# Autodesk Inventor assembly: Сборка всего
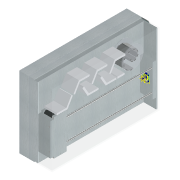
[picture p0: Inventor's stored thumbnail of the model, 180x180]
Saved by Autodesk Inventor 2022 (Build 260153000, 153)
## iProperties
Created: 2023-02-18
Part Number: Сборка всего
Document SubType Name: Assembly
Designer: Глеб
Mass: 16857.9 g
Surface Area: 28110.4 cm^2
Volume: 16853.6 cm^3
Density: 1.00025 g/cm^3
Author: Глеб
## Documents named in this file (12)
- C:\Users\Глеб\Documents\Inventor\Файлы Inventor\Сборка всего.iam
- C:\Users\Глеб\Documents\Inventor\Файлы Inventor\Общий концепт в 3д.ipt
- C:\Users\Глеб\Documents\Inventor\Файлы Inventor\Барабан сборка.iam
- C:\Users\Глеб\Documents\Inventor\Файлы Inventor\Лепестки со шпильками сборка.iam
- C:\Users\Глеб\Documents\Inventor\Файлы Inventor\Конвейр сборка.iam
- C:\Users\Глеб\Documents\Inventor\Файлы Inventor\Стенка БСП.iam
- C:\Users\Глеб\Documents\Inventor\Файлы Inventor\Стеклянная крышка.ipt
- C:\Users\Глеб\Documents\Inventor\Файлы Inventor\Механизм подъема.iam
- C:\Users\Глеб\Documents\Inventor\Файлы Inventor\Задняя стенка.ipt
- C:\Users\Глеб\Documents\Inventor\Файлы Inventor\Крепления и направляющие.iam
- C:\Users\Глеб\Documents\Inventor\Файлы Inventor\28BYJ-48 мотор.ipt
- C:\Users\Глеб\Documents\Inventor\Файлы Inventor\XPT2046 Touch Controller.ipt
## Components (16 placed, 11 different names)
1. Общий концепт в 3д:1 — Совмещение:47, Совмещение:48, Заподлицо:12, Совмещение:52, Совмещение:58, Совмещение:60, Заподлицо:64, Заподлицо:65, Совмещение:62, Заподлицо:66, Совмещение:64, Совмещение:65, Заподлицо:73, Заподлицо:74
2. Барабан сборка:1 [sub-assembly] — Совмещение:47, Совмещение:50, Совмещение:51
3. Лепестки со шпильками сборка:1 [sub-assembly] — Угол:1, Угол:2, Совмещение:48, Заподлицо:1, Заподлицо:4, Заподлицо:6, Заподлицо:7, Совмещение:49, Заподлицо:8, Заподлицо:12, Симметрия:1
4. Лепестки со шпильками сборка:5 [sub-assembly] — Угол:3, Угол:4, Заподлицо:2, Заподлицо:7, Совмещение:49, Заподлицо:8, Заподлицо:9, Симметрия:1, Заподлицо:14, Совмещение:54
5. Лепестки со шпильками сборка:6 [sub-assembly] — Заподлицо:1, Заподлицо:3, Заподлицо:5, Заподлицо:9, Заподлицо:10
6. Лепестки со шпильками сборка:7 [sub-assembly] — Заподлицо:2, Заподлицо:6, Заподлицо:10, Заподлицо:11
7. Лепестки со шпильками сборка:8 [sub-assembly] — Заподлицо:3, Заподлицо:4, Заподлицо:5, Заподлицо:11, Совмещение:59
8. Стенка БСП:1 [sub-assembly] — Заподлицо:14, Совмещение:52, Совмещение:54, Заподлицо:16, Угол:5
9. Конвейр сборка:1 [sub-assembly] — Совмещение:66, Заподлицо:67, Совмещение:67, Совмещение:68
10. Стеклянная крышка:1
11. Лепестки со шпильками сборка:9 [sub-assembly] — Угол:5, Совмещение:58, Совмещение:59, Совмещение:66, Заподлицо:67
12. Задняя стенка:1 — Совмещение:60, Заподлицо:64, Заподлицо:65, Совмещение:69, Заподлицо:68, Заподлицо:72, Заподлицо:73, Заподлицо:74
13. Крепления и направляющие:1 [sub-assembly] — Совмещение:62, Заподлицо:66, Совмещение:67
14. 28BYJ-48 мотор:1 — Совмещение:64, Совмещение:65
15. Механизм подъема:1 [sub-assembly] — Совмещение:68, Совмещение:69
16. XPT2046 Touch Controller:1 — Совмещение:70, Заподлицо:72
## Relationships (47: Flush 23, Mate 18, Angle 5, Symmetry 1)
- Совмещение:47 [Mate]: Общий концепт в 3д:1 ↔ Барабан сборка:1
- Угол:1 [Angle] (0 deg): Лепестки со шпильками сборка:1
- Угол:2 [Angle] (0 deg): Лепестки со шпильками сборка:1
- Совмещение:48 [Mate]: Общий концепт в 3д:1 ↔ Лепестки со шпильками сборка:1
- Угол:3 [Angle] (0 deg): Лепестки со шпильками сборка:5
- Угол:4 [Angle] (180 deg): Лепестки со шпильками сборка:5
- Заподлицо:1 [Flush]: Лепестки со шпильками сборка:1 ↔ Лепестки со шпильками сборка:6
- Заподлицо:2 [Flush]: Лепестки со шпильками сборка:5 ↔ Лепестки со шпильками сборка:7
- Заподлицо:3 [Flush]: Лепестки со шпильками сборка:6 ↔ Лепестки со шпильками сборка:8
- Заподлицо:4 [Flush]: Лепестки со шпильками сборка:1 ↔ Лепестки со шпильками сборка:8
- Заподлицо:5 [Flush]: Лепестки со шпильками сборка:6 ↔ Лепестки со шпильками сборка:8
- Заподлицо:6 [Flush]: Лепестки со шпильками сборка:1 ↔ Лепестки со шпильками сборка:7
- Заподлицо:7 [Flush]: Лепестки со шпильками сборка:1 ↔ Лепестки со шпильками сборка:5
- Совмещение:49 [Mate] (-100 mm): Лепестки со шпильками сборка:1 ↔ Лепестки со шпильками сборка:5
- Заподлицо:8 [Flush] (-50 mm): Лепестки со шпильками сборка:1 ↔ Лепестки со шпильками сборка:5
- Заподлицо:9 [Flush] (-50 mm): Лепестки со шпильками сборка:5 ↔ Лепестки со шпильками сборка:6
- Заподлицо:10 [Flush] (-50 mm): Лепестки со шпильками сборка:6 ↔ Лепестки со шпильками сборка:7
- Заподлицо:11 [Flush] (-50 mm): Лепестки со шпильками сборка:7 ↔ Лепестки со шпильками сборка:8
- Заподлицо:12 [Flush] (40 mm): Общий концепт в 3д:1 ↔ Лепестки со шпильками сборка:1
- Симметрия:1 [Symmetry]: Лепестки со шпильками сборка:1 ↔ Лепестки со шпильками сборка:5
- Совмещение:50 [Mate]: Барабан сборка:1
- Заподлицо:13 [Flush] (-14 mm)
- Совмещение:51 [Mate]: Барабан сборка:1
- Заподлицо:14 [Flush]: Лепестки со шпильками сборка:5 ↔ Стенка БСП:1
- Совмещение:52 [Mate]: Общий концепт в 3д:1 ↔ Стенка БСП:1
- Совмещение:54 [Mate] (5 mm): Лепестки со шпильками сборка:5 ↔ Стенка БСП:1
- Заподлицо:16 [Flush] (70 mm): Стенка БСП:1
- Угол:5 [Angle] (60 deg): Стенка БСП:1 ↔ Лепестки со шпильками сборка:9
- Совмещение:58 [Mate]: Общий концепт в 3д:1 ↔ Лепестки со шпильками сборка:9
- Совмещение:59 [Mate] (5 mm): Лепестки со шпильками сборка:8 ↔ Лепестки со шпильками сборка:9
- Совмещение:60 [Mate]: Общий концепт в 3д:1 ↔ Задняя стенка:1
- Заподлицо:64 [Flush]: Общий концепт в 3д:1 ↔ Задняя стенка:1
- Заподлицо:65 [Flush]: Общий концепт в 3д:1 ↔ Задняя стенка:1
- Совмещение:62 [Mate]: Общий концепт в 3д:1 ↔ Крепления и направляющие:1
- Заподлицо:66 [Flush]: Общий концепт в 3д:1 ↔ Крепления и направляющие:1
- Совмещение:64 [Mate]: Общий концепт в 3д:1 ↔ 28BYJ-48 мотор:1
- Совмещение:65 [Mate]: Общий концепт в 3д:1 ↔ 28BYJ-48 мотор:1
- Совмещение:66 [Mate] (1 mm): Конвейр сборка:1 ↔ Лепестки со шпильками сборка:9
- Заподлицо:67 [Flush]: Конвейр сборка:1 ↔ Лепестки со шпильками сборка:9
- Совмещение:67 [Mate]: Конвейр сборка:1 ↔ Крепления и направляющие:1
- Совмещение:68 [Mate]: Конвейр сборка:1 ↔ Механизм подъема:1
- Совмещение:69 [Mate] (1 mm): Задняя стенка:1 ↔ Механизм подъема:1
- Заподлицо:68 [Flush]: Задняя стенка:1
- Совмещение:70 [Mate]: XPT2046 Touch Controller:1
- Заподлицо:72 [Flush] (17 mm): Задняя стенка:1 ↔ XPT2046 Touch Controller:1
- Заподлицо:73 [Flush]: Общий концепт в 3д:1 ↔ Задняя стенка:1
- Заподлицо:74 [Flush]: Общий концепт в 3д:1 ↔ Задняя стенка:1
